# Autodesk Inventor assembly: Display_Assembly
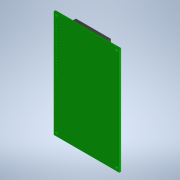
[picture p0: Inventor's stored thumbnail of the model, 180x180]
Saved by Autodesk Inventor 2020 (Build 240168000, 168)
## iProperties
Created: 2020-11-23
Part Number: Display_Assembly
Document SubType Name: Assembly
Designer: nico
Author: nico
## Documents named in this file (3)
- Y:\Technik\Technik 2020\04 - Electronics\Altium-libs-fix\libs\libNico\EA_W204-XLG\Display_Assembly.iam
- Y:\Technik\Technik 2020\04 - Electronics\Altium-libs-fix\libs\libNico\EA_W204-XLG\Display.ipt
- Y:\Technik\Technik 2020\04 - Electronics\Altium-libs-fix\libs\libNico\EA_W204-XLG\Mounting_PCB.ipt
## Components (2 placed, 2 different names)
1. Display:1 — Mate:1, Flush:1, Flush:2
2. Mounting_PCB:1 — Mate:1, Flush:1, Flush:2
## Relationships (3: Flush 2, Mate 1)
- Mate:1: Display:1 ↔ Mounting_PCB:1
- Flush:1 (2 mm): Display:1 ↔ Mounting_PCB:1
- Flush:2 (14 mm): Display:1 ↔ Mounting_PCB:1
